# Autodesk Inventor assembly: 2f2
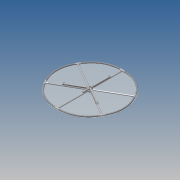
[picture p0: Inventor's stored thumbnail of the model, 180x180]
Saved by Autodesk Inventor 2014 SP1 (Build 180222100, 222)
## iProperties
Company: HERA Project
Created: 2013-06-27
Part Number: 2f2
Document SubType Name: Assembly
Designer: David DeBoer
Description: Feed backplane support assembly
Author: David DeBoer
Title: Feed backplane support
## Documents named in this file (11)
- C:\Users\Dave\Desktop\hera-cad\feed\bpSupAssembly.iam
- C:\Users\Dave\Desktop\hera-cad\feed\bpSupCross.ipt
- C:\Users\Dave\Desktop\hera-cad\feed\bpSupInner1.ipt
- C:\Users\Dave\Desktop\hera-cad\feed\collar.ipt
- C:\Users\Dave\Desktop\hera-cad\feed\bpSupArm.ipt
- C:\Users\Dave\Desktop\hera-cad\smallParts\eyebolt_ss_375.ipt
- C:\Users\Dave\Desktop\hera-cad\smallParts\nut_ss_375.ipt
- C:\Users\Dave\Desktop\hera-cad\smallParts\pvc_T_0.75in.ipt
- C:\Users\Dave\Desktop\hera-cad\feed\bpSupArc.ipt
- C:\Users\Dave\Desktop\hera-cad\feed\bpScreen.ipt
- C:\Users\Dave\Desktop\hera-cad\smallParts\D.ipt
## Components (28 placed, 10 different names)
1. bpSupCross:1 — Mate:3, Insert:1, Insert:2, Insert:7, Mate:4, Flush:1, Flush:2, Insert:8
2. bpSupInner1:2 — Mate:3, Flush:2
3. collar:1 — Insert:1, Insert:6
4. eyebolt_ss_375:1 — Insert:2, Insert:3
5. nut_ss_375:1 — Insert:3
6. bpScreen:1 — Insert:6
7. bpSupInner1:3 — Mate:4, Flush:1
8. bpSupArm:1 — Insert:4
9. bpSupArm:2
10. bpSupArm:3
11. bpSupArm:4
12. bpSupArm:5
13. bpSupArm:6
14. pvc_T_0.75in:1 — Insert:4, Insert:5
15. pvc_T_0.75in:2
16. pvc_T_0.75in:3
17. pvc_T_0.75in:4
18. pvc_T_0.75in:5
19. pvc_T_0.75in:6
20. bpSupArc:1 — Insert:5
21. bpSupArc:2
22. bpSupArc:3
23. bpSupArc:4
24. bpSupArc:5
25. bpSupArc:6
26. D:1 — Insert:7, Insert:8
27. D:2
28. D:3
## Component patterns: arms (6 elements), Ts (6 elements), (6 elements, first: bpSupArc:1), (3 elements, first: D:1)
## Relationships (12: Insert 8, Mate 2, Flush 2)
- Mate:3: bpSupCross:1 ↔ bpSupInner1:2
- Insert:1: bpSupCross:1 ↔ collar:1
- Insert:2 (-50.8 mm): bpSupCross:1 ↔ eyebolt_ss_375:1
- Insert:3 (-12.7 mm): eyebolt_ss_375:1 ↔ nut_ss_375:1
- Insert:4 (-12.7 mm): bpSupArm:1 ↔ pvc_T_0.75in:1
- Insert:5: pvc_T_0.75in:1 ↔ bpSupArc:1
- Insert:6 (-25.4 mm): collar:1 ↔ bpScreen:1
- Insert:7 (-34.29 mm): bpSupCross:1 ↔ D:1
- Mate:4: bpSupCross:1 ↔ bpSupInner1:3
- Flush:1: bpSupCross:1 ↔ bpSupInner1:3
- Flush:2: bpSupCross:1 ↔ bpSupInner1:2
- Insert:8 (-7.62 mm): bpSupCross:1 ↔ D:1
